# Autodesk Inventor assembly: tarot_5008_340kv_assy
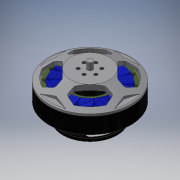
[picture p0: Inventor's stored thumbnail of the model, 180x180]
Saved by Autodesk Inventor 2019.4 (Build 234330000, 330)
## iProperties
Created: 2019-10-01
Part Number: tarot_5008_340kv_assy
Document SubType Name: Assembly
Designer: cdi
Author: cdi
## Documents named in this file (8)
- D:\SynologyDrive\workspace_inventor\2019_06_19.MT4008_actuator\tarot_5008_340kv\tarot_5008_340kv_assy.iam
- D:\SynologyDrive\workspace_inventor\2019_06_19.MT4008_actuator\tarot_5008_340kv\housing0.ipt
- D:\SynologyDrive\workspace_inventor\2019_06_19.MT4008_actuator\tarot_5008_340kv\housing1.ipt
- D:\SynologyDrive\workspace_inventor\2019_06_19.MT4008_actuator\tarot_5008_340kv\arc_magnet_10_10_2.ipt
- D:\SynologyDrive\workspace_inventor\2019_06_19.MT4008_actuator\tarot_5008_340kv\stator.ipt
- D:\SynologyDrive\workspace_inventor\2019_06_19.MT4008_actuator\tarot_5008_340kv\core.ipt
- D:\SynologyDrive\workspace_inventor\2019_06_19.MT4008_actuator\tarot_5008_340kv\bearing_6_12_3.ipt
- D:\SynologyDrive\workspace_inventor\2019_06_19.MT4008_actuator\tarot_5008_340kv\winding.ipt
## Components (131 placed, 7 different names)
1. housing0:1 — Mate:1, Mate:3, Mate:5, Mate:7, Mate:8, Flush:3
2. housing1:1 — Mate:2, Mate:3, Mate:6
3. stator:1 — Mate:7, Flush:1, Flush:2, Mate:10, Mate:11
4. core:1 — Mate:8, Flush:2, Mate:9
5. bearing_6_12_3:1 — Mate:9, Flush:3
6. arc_magnet_10_10_2:1 — Mate:5, Mate:6, Angle:1
7. arc_magnet_10_10_2:2
8. arc_magnet_10_10_2:3
9. arc_magnet_10_10_2:4
10. arc_magnet_10_10_2:5 — Flush:1
11. arc_magnet_10_10_2:6
12. arc_magnet_10_10_2:7
13. arc_magnet_10_10_2:8
14. arc_magnet_10_10_2:9
15. arc_magnet_10_10_2:10
16. arc_magnet_10_10_2:11
17. arc_magnet_10_10_2:12
18. arc_magnet_10_10_2:13
19. arc_magnet_10_10_2:14
20. winding:1 — Mate:10, Mate:11
21. winding:2
22. winding:3
23. winding:4
24. winding:5
25. winding:6
26. winding:7
27. winding:8
28. winding:9
29. winding:10
30. winding:11
31. winding:12
32. winding:13
33. winding:14
34. winding:15
35. winding:16
36. winding:17
37. winding:18
38. winding:19
39. winding:20
40. winding:21
41. winding:22
42. winding:23
43. winding:24
44. winding:25
45. winding:26
46. winding:27
47. winding:28
48. winding:29
49. winding:30
50. winding:31
51. winding:32
52. winding:33
53. winding:34
54. winding:35
55. winding:36
56. winding:37
57. winding:38
58. winding:39
59. winding:40
60. winding:41
61. winding:42
62. winding:43
63. winding:44
64. winding:45
65. winding:46
66. winding:47
67. winding:48
68. winding:49
69. winding:50
70. winding:51
71. winding:52
72. winding:53
73. winding:54
74. winding:55
75. winding:56
76. winding:57
77. winding:58
78. winding:59
79. winding:60
80. winding:61
81. winding:62
82. winding:63
83. winding:64
84. winding:65
85. winding:66
86. winding:67
87. winding:68
88. winding:69
89. winding:70
90. winding:71
91. winding:72
92. winding:73
93. winding:74
94. winding:75
95. winding:76
96. winding:77
97. winding:78
98. winding:79
99. winding:80
100. winding:81
101. winding:82
102. winding:83
103. winding:84
104. winding:85
105. winding:86
106. winding:87
107. winding:88
108. winding:89
109. winding:90
110. winding:91
111. winding:92
112. winding:93
113. winding:94
114. winding:95
115. winding:96
116. winding:97
117. winding:98
118. winding:99
119. winding:100
120. winding:101
121. winding:102
122. winding:103
123. winding:104
124. winding:105
125. winding:106
126. winding:107
127. winding:108
128. winding:109
129. winding:110
130. winding:111
131. winding:112
## Component patterns: (14 elements, first: arc_magnet_10_10_2:1), (14 elements), (8 elements, first: winding:1), Component Pattern 2:2 (8 elements), Component Pattern 2:3 (8 elements), Component Pattern 2:4 (8 elements), Component Pattern 2:5 (8 elements), Component Pattern 2:6 (8 elements), Component Pattern 2:7 (8 elements), Component Pattern 2:8 (8 elements), Component Pattern 2:9 (8 elements), Component Pattern 2:10 (8 elements), Component Pattern 2:11 (8 elements), Component Pattern 2:12 (8 elements), Component Pattern 2:13 (8 elements), Component Pattern 2:14 (8 elements)
## Relationships (14: Mate 10, Flush 3, Angle 1)
- Mate:1: housing0:1
- Mate:2: housing1:1
- Mate:3: housing0:1 ↔ housing1:1
- Mate:5: housing0:1 ↔ arc_magnet_10_10_2:1
- Mate:6: housing1:1 ↔ arc_magnet_10_10_2:1
- Angle:1 (0 deg): arc_magnet_10_10_2:1
- Mate:7: housing0:1 ↔ stator:1
- Flush:1: stator:1 ↔ arc_magnet_10_10_2:5
- Mate:8: housing0:1 ↔ core:1
- Flush:2: stator:1 ↔ core:1
- Mate:9: core:1 ↔ bearing_6_12_3:1
- Flush:3: housing0:1 ↔ bearing_6_12_3:1
- Mate:10: stator:1 ↔ winding:1
- Mate:11: stator:1 ↔ winding:1
